# Autodesk Inventor assembly: Case_and_Lid
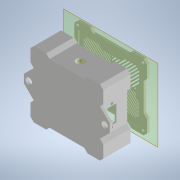
[picture p0: Inventor's stored thumbnail of the model, 180x180]
Saved by Autodesk Inventor 2020 (Build 240168000, 168)
## iProperties
Created: 2020-03-10
Part Number: Case_and_Lid
Document SubType Name: Assembly
Designer: Alex
Author: Alex
## Documents named in this file (3)
- C:\Users\Alex\Documents\Inventor\Ventolino_Nano\Case_and_Lid.iam
- C:\Users\Alex\Documents\Inventor\Ventolino_Nano\Case.ipt
- C:\Users\Alex\Documents\Inventor\Ventolino_Nano\Lid.ipt
## Components (2 placed, 2 different names)
1. Case:1 — Flush:1
2. Lid:1 — Flush:2
## Relationships (2: Flush 2)
- Flush:1 (20 mm): Case:1
- Flush:2: Lid:1
